# Autodesk Inventor assembly: Assembly
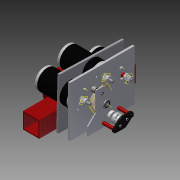
[picture p0: Inventor's stored thumbnail of the model, 180x180]
Saved by Autodesk Inventor 2013 (Build 170138000, 138)
## iProperties
Created: 2013-06-04
Part Number: Assembly
Document SubType Name: Assembly
Designer: mvarma
Author: mvarma
## Documents named in this file (55)
- C:\Users\mvarma\Desktop\GRT 2013-2014 Gearbox\Mark 2\Assembly.iam
- C:\Users\mvarma\Desktop\GRT 2013-2014 Gearbox\Mark 2\Frame Segment.ipt
- C:\Users\mvarma\Desktop\GRT 2013-2014 Gearbox\Mark 2\Plates\Cim Plate.ipt
- C:\Users\mvarma\Desktop\GRT 2013-2014 Gearbox\Mark 2\Wheel Temp.ipt
- C:\Users\mvarma\Desktop\GRT 2013-2014 Gearbox\Mark 2\Motors\Mini CIM Motor.ipt
- C:\Users\mvarma\Desktop\GRT 2013-2014 Gearbox\Mark 2\Motors\CIM Motor.ipt
- C:\Users\mvarma\Desktop\GRT 2013-2014 Gearbox\Mark 2\Pulleys\16T 3mm GT2 - 8mm Key Broach.ipt
- C:\Users\mvarma\Desktop\GRT 2013-2014 Gearbox\Mark 2\Pulleys\48T 3mm GT2 - .375 Hex Broach - Hubless.ipt
- C:\Users\mvarma\Desktop\GRT 2013-2014 Gearbox\Mark 2\Pulleys\56T 3mm GT2 - .375 Hex Broach - Hubless.ipt
- C:\Users\mvarma\Desktop\GRT 2013-2014 Gearbox\Mark 2\Bearings\FR6-2ZZ - Hex.ipt
- C:\Users\mvarma\Desktop\GRT 2013-2014 Gearbox\Mark 2\Spacers\Shim 10 thou .500 Bore.ipt
- C:\Users\mvarma\Desktop\GRT 2013-2014 Gearbox\Mark 2\Shafts\Belt Shaft.ipt
- C:\Users\mvarma\Desktop\GRT 2013-2014 Gearbox\Mark 2\.2500 Spring Clip.ipt
- C:\Users\mvarma\Desktop\GRT 2013-2014 Gearbox\Mark 2\Bearings\R4-2RS.ipt
- C:\Users\mvarma\Desktop\GRT 2013-2014 Gearbox\Mark 2\Spacers\Belt Shaft Spacer 1.ipt
- C:\Users\mvarma\Desktop\GRT 2013-2014 Gearbox\Mark 2\Plates\Pnuematic Plate.ipt
- C:\Users\mvarma\Desktop\GRT 2013-2014 Gearbox\Mark 2\Spacers\Shim 10 thou .375 Bore.ipt
- C:\Users\mvarma\Desktop\GRT 2013-2014 Gearbox\Mark 2\Bearings\FR6-2RS.ipt
- C:\Users\mvarma\Desktop\GRT 2013-2014 Gearbox\Mark 2\Spacers\Belt Shaft Spacer 2.ipt
- C:\Users\mvarma\Desktop\GRT 2013-2014 Gearbox\Mark 2\Shafts\Cluster Shaft.ipt
- C:\Users\mvarma\Desktop\GRT 2013-2014 Gearbox\Mark 2\Gears\15T 20DP - .375 Hex Bore.ipt
- C:\Users\mvarma\Desktop\GRT 2013-2014 Gearbox\Mark 2\Gears\28T 20DP - .375 Hex Bore.ipt
- C:\Users\mvarma\Desktop\GRT 2013-2014 Gearbox\Mark 2\Bearings\FR8-2RS.ipt
- C:\Users\mvarma\Desktop\GRT 2013-2014 Gearbox\Mark 2\Spacers\MiniCim Spacer.ipt
- C:\Users\mvarma\Desktop\GRT 2013-2014 Gearbox\Mark 2\Spacers\Cim Spacer.ipt
- C:\Users\mvarma\Desktop\GRT 2013-2014 Gearbox\Mark 2\Plates\Mounting Plate.ipt
- C:\Users\mvarma\Desktop\GRT 2013-2014 Gearbox\Mark 2\Gears\35T 20DP - .188 Ball Shifting Bore.ipt
- C:\Users\mvarma\Desktop\GRT 2013-2014 Gearbox\Mark 2\Gears\48T 20DP - .188 Ball Shifting Bore.ipt
- C:\Users\mvarma\Desktop\GRT 2013-2014 Gearbox\Mark 2\Bearings\Thrust Bearing Washer - .6250 Bore.ipt
- C:\Users\mvarma\Desktop\GRT 2013-2014 Gearbox\Mark 2\Spacers\Cluster Shaft Spacer.ipt
- C:\Users\mvarma\Desktop\GRT 2013-2014 Gearbox\Mark 2\Bearings\R10-Open.ipt
- C:\Users\mvarma\Desktop\GRT 2013-2014 Gearbox\Mark 2\Bearings\R10-2RS.ipt
- C:\Users\mvarma\Desktop\GRT 2013-2014 Gearbox\Mark 2\Bearing Cover.ipt
- C:\Users\mvarma\Desktop\GRT 2013-2014 Gearbox\Mark 2\Shafts\Output Shaft.ipt
- C:\Users\mvarma\Desktop\GRT 2013-2014 Gearbox\Mark 2\Shafts\Shifting Shaft.ipt
- C:\Users\mvarma\Desktop\GRT 2013-2014 Gearbox\Mark 2\Shafts\Output Shaft Insert.ipt
- C:\Users\mvarma\Desktop\GRT 2013-2014 Gearbox\Mark 2\Ball Bearing 3- 16  in .ipt
- C:\Users\mvarma\Desktop\GRT 2013-2014 Gearbox\Mark 2\Pneumatic\Bore.ipt
- C:\Users\mvarma\Desktop\GRT 2013-2014 Gearbox\Mark 2\Pneumatic\Cylinder.ipt
- C:\Users\mvarma\Desktop\GRT 2013-2014 Gearbox\Mark 2\Pneumatic\Front Mount.ipt
- C:\Users\mvarma\Desktop\GRT 2013-2014 Gearbox\Mark 2\Pneumatic\Rear Mount.ipt
- C:\Users\mvarma\Desktop\GRT 2013-2014 Gearbox\Mark 2\Pneumatic\Shaft.ipt
- C:\Users\mvarma\Desktop\GRT 2013-2014 Gearbox\Mark 2\Pneumatic\Spacer.ipt
- C:\Users\mvarma\Desktop\GRT 2013-2014 Gearbox\Mark 2\Bolts\Socket Head Cap Screw 8-32 Thread .375 Length.ipt
- C:\Users\mvarma\Desktop\GRT 2013-2014 Gearbox\Mark 2\Bolts\Button Head Cap Screw 6-32 Thread .250 Length.ipt
- C:\Users\mvarma\Desktop\GRT 2013-2014 Gearbox\Mark 2\Pneumatic\Pneumatic Connector - Side Side.ipt
- C:\Users\mvarma\Desktop\GRT 2013-2014 Gearbox\Mark 2\Pneumatic\Pneumatic Connector -Actuator Side.ipt
- C:\Users\mvarma\Desktop\GRT 2013-2014 Gearbox\Mark 2\Bolts\Socket Head Cap Screw 8-32 Thread .750 Length.ipt
- C:\Users\mvarma\Desktop\GRT 2013-2014 Gearbox\Mark 2\Bolts\Socket Head Cap Screw 4-40 Thread 1.000 Length.ipt
- C:\Users\mvarma\Desktop\GRT 2013-2014 Gearbox\Mark 2\Spring Pin 1-16 Diameter.ipt
- C:\Users\mvarma\Desktop\GRT 2013-2014 Gearbox\Mark 2\Pneumatic\Mouning Standoff.ipt
- C:\Users\mvarma\Desktop\GRT 2013-2014 Gearbox\Mark 2\Pneumatic\Mounting Insert.ipt
- C:\Users\mvarma\Desktop\GRT 2013-2014 Gearbox\Mark 2\Plates\Pneumatic Mounting Plate.ipt
- C:\Users\mvarma\Desktop\GRT 2013-2014 Gearbox\Mark 2\Pem Nuts\4-40 Clinch Style Pem Nut .091 Minimum Panel Thickness.ipt
- C:\Users\mvarma\Desktop\GRT 2013-2014 Gearbox\Mark 2\Bolts\Socket Head Cap Screw 10-32 Thread 3.000 Length.ipt
## Components (81 placed, 54 different names)
1. Frame Segment:1 — Mate:1, Angle:1, Mate:2, Mate:70, Mate:71
2. Wheel Temp:1 — Mate:2
3. .2500 Spring Clip:1 — Mate:25, Mate:26
4. .2500 Spring Clip:2 — Mate:39, Mate:40
5. Cluster Shaft Spacer:1 — Mate:100, Mate:101
6. R10-2RS:1 — Mate:102, Flush:12
7. Bearing Cover:1 — Mate:106, Mate:107, Mate:108, Mate:160, Mate:161, Mate:162, Mate:163
8. Socket Head Cap Screw 10-32 Thread 3.000 Length:1 — Mate:175, Mate:176
9. Socket Head Cap Screw 10-32 Thread 3.000 Length:2 — Mate:173, Mate:174
10. FR6-2RS:2 — Mate:74, Mate:75, Mate:101
11. FR8-2RS:2 — Mate:72, Mate:73, Mate:99, Flush:13
12. R10-Open:1 — Mate:76, Mate:77, Mate:80, Mate:92, Mate:97, Mate:98
13. R10-Open:2 — Mate:78, Mate:79, Mate:81, Flush:11, Mate:104, Mate:105
14. FR6-2RS:1 — Mate:36, Mate:37, Mate:38, Flush:10
15. FR6-2ZZ - Hex:1 — Mate:19, Mate:20, Angle:3, Mate:22, Mate:44, Mate:96
16. R4-2RS:1 — Mate:27, Mate:28, Mate:29, Flush:9
17. R4-2RS:2 — Mate:27, Mate:28, Mate:42
18. Pneumatic Mounting Plate:1 — Mate:166, Mate:167, Mate:168, Mate:169, Mate:170, Mate:171, Mate:172, Mate:173, Mate:174, Mate:175, Mate:176
19. Mounting Plate:1 — Mate:70, Mate:71, Mate:72, Mate:73, Mate:74, Mate:75
20. Pnuematic Plate:1 — Mate:32, Mate:33, Mate:34, Mate:36, Mate:37, Mate:43
21. Cim Plate:1 — Mate:1, Angle:1, Mate:3, Mate:4, Mate:5, Mate:6, Mate:7, Mate:8, Mate:9, Mate:10, Mate:11, Mate:15, Mate:16, Mate:19, Mate:20, Mate:21, Mate:24, Flush:8, Mate:31, Mate:32, Mate:33, Mate:45, Mate:46, Mate:80, Mate:81, Mate:102, Flush:12, Mate:106, Mate:107, Mate:108, Mate:111
22. 16T 3mm GT2 - 8mm Key Broach:1 — Mate:13, Flush:5, Flush:6
23. 16T 3mm GT2 - 8mm Key Broach:2 — Mate:12, Flush:4, Flush:7
24. 16T 3mm GT2 - 8mm Key Broach:3 — Mate:14, Flush:3, Mate:18
25. 48T 3mm GT2 - .375 Hex Broach - Hubless:1 — Mate:15, Mate:17, Angle:2, Flush:6, Flush:7, Mate:23, Flush:9
26. 56T 3mm GT2 - .375 Hex Broach - Hubless:1 — Mate:16, Mate:17, Angle:2, Mate:18, Angle:3, Mate:35
27. Mini CIM Motor:1 — Mate:3, Mate:4, Mate:5, Mate:14, Flush:3, Mate:51, Mate:52
28. CIM Motor:1 — Mate:9, Mate:10, Mate:11, Mate:12, Flush:4, Mate:53, Mate:54
29. CIM Motor:2 — Mate:6, Mate:7, Mate:8, Mate:13, Flush:5, Mate:55, Mate:56
30. Belt Shaft Spacer 1:1 — Mate:30, Mate:31
31. Belt Shaft Spacer 2:1 — Mate:41, Mate:42
32. MiniCim Spacer:1 — Mate:51, Mate:52
33. Cim Spacer:1 — Mate:53, Mate:54
34. Cim Spacer:2 — Mate:55, Mate:56
35. Shim 10 thou .375 Bore:1 — Mate:34, Mate:35, Mate:38
36. Shim 10 thou .500 Bore:1 — Mate:21, Mate:22, Mate:23
37. Shim 10 thou .500 Bore:2 — Mate:97, Mate:98, Mate:99
38. Thrust Bearing Washer - .6250 Bore:1 — Mate:90, Mate:91, Mate:94
39. Thrust Bearing Washer - .6250 Bore:2 — Mate:90, Mate:91, Mate:92, Mate:93
40. Thrust Bearing Washer - .6250 Bore:3 — Mate:104, Mate:105
41. Belt Shaft:1 — Mate:24, Mate:25, Mate:26, Flush:8, Mate:29, Mate:30, Mate:39, Mate:40, Mate:41
42. Cluster Shaft:1 — Mate:43, Flush:10, Mate:44, Angle:4, Mate:100
43. Output Shaft:1 — Mate:109, Mate:110, Mate:111, Flush:13, Mate:112, Mate:113, Mate:114, Mate:115, Mate:116, Mate:117, Mate:118, Mate:119
44. Shifting Shaft:1 — Mate:109, Mate:110, Transitional:1, Transitional:2, Transitional:3, Transitional:4, Transitional:5, Transitional:6, Mate:135, Flush:16, Mate:158, Flush:17
45. Output Shaft Insert:1 — Mate:112, Mate:113
46. 15T 20DP - .375 Hex Bore:1 — Mate:45, Angle:4, Angle:5, Flush:11, Mate:95, Mate:96
47. 28T 20DP - .375 Hex Bore:1 — Mate:46, Angle:5, Mate:95
48. 35T 20DP - .188 Ball Shifting Bore:1 — Mate:76, Mate:77, Mate:94
49. 48T 20DP - .188 Ball Shifting Bore:1 — Mate:78, Mate:79, Mate:93
50. Ball Bearing 3- 16  in :1 — Mate:116, Transitional:2
51. Ball Bearing 3- 16  in :2 — Mate:114, Transitional:6
52. Ball Bearing 3- 16  in :3 — Mate:115, Transitional:5
53. Ball Bearing 3- 16  in :4 — Mate:117, Transitional:4
54. Ball Bearing 3- 16  in :5 — Mate:119, Transitional:3
55. Ball Bearing 3- 16  in :6 — Mate:118, Transitional:1
56. Bore:1 — Mate:133, Flush:14, Flush:15
57. Cylinder:1 — Mate:130, Mate:131, Mate:132, Flush:15
58. Front Mount:1 — Mate:128, Mate:129, Mate:134, Mate:135, Mate:154, Mate:155, Mate:156, Mate:157
59. Rear Mount:1 — Mate:120, Mate:121, Mate:122, Mate:123, Mate:124, Mate:125, Mate:126, Mate:127, Mate:130, Mate:131, Flush:18, Mate:164, Mate:165, Flush:19, Flush:20, Mate:167
60. Shaft:1 — Mate:132, Mate:133, Flush:14, Mate:138, Mate:139, Mate:140
61. Spacer:1 — Mate:120, Mate:124
62. Spacer:2 — Mate:121, Mate:125, Mate:128
63. Spacer:3 — Mate:122, Mate:126
64. Spacer:4 — Mate:123, Mate:127, Mate:129, Mate:134
65. Socket Head Cap Screw 4-40 Thread 1.000 Length:1 — Mate:155, Mate:157
66. Socket Head Cap Screw 4-40 Thread 1.000 Length:2 — Mate:154, Mate:156
67. Spring Pin 1-16 Diameter:1 — Mate:158, Flush:17
68. Mouning Standoff:1 — Mate:160, Mate:161, Mate:166, Mate:168
69. Mouning Standoff:2 — Mate:162, Mate:163, Flush:18
70. Mounting Insert:1 — Mate:164, Flush:20
71. Mounting Insert:2 — Mate:165, Flush:19
72. 4-40 Clinch Style Pem Nut .091 Minimum Panel Thickness:1 — Mate:169, Mate:170
73. 4-40 Clinch Style Pem Nut .091 Minimum Panel Thickness:2 — Mate:171, Mate:172
74. Socket Head Cap Screw 8-32 Thread .750 Length:2 — Mate:145, Mate:146
75. Socket Head Cap Screw 8-32 Thread .375 Length:1 — Mate:136, Mate:137
76. Button Head Cap Screw 6-32 Thread .250 Length:1 — Mate:152, Mate:153
77. Button Head Cap Screw 6-32 Thread .250 Length:2 — Mate:150, Mate:151
78. Socket Head Cap Screw 8-32 Thread .750 Length:1 — Mate:144, Mate:147
79. R4-2RS:3 — Mate:148, Mate:149, Flush:16
80. Pneumatic Connector - Side Side:1 — Mate:141, Mate:142, Mate:143, Mate:148, Mate:149, Mate:150, Mate:151, Mate:152, Mate:153
81. Pneumatic Connector -Actuator Side:1 — Mate:136, Mate:137, Mate:138, Mate:139, Mate:140, Mate:141, Mate:142, Mate:143, Mate:144, Mate:145, Mate:146, Mate:147
## Relationships (178: Mate 149, Flush 18, Transitional 6, Angle 5)
- Mate:1: Frame Segment:1 ↔ Cim Plate:1
- Angle:1 (0 deg): Frame Segment:1 ↔ Cim Plate:1
- Mate:2: Frame Segment:1 ↔ Wheel Temp:1
- Mate:3: Cim Plate:1 ↔ Mini CIM Motor:1
- Mate:4: Cim Plate:1 ↔ Mini CIM Motor:1
- Mate:5: Cim Plate:1 ↔ Mini CIM Motor:1
- Mate:6: Cim Plate:1 ↔ CIM Motor:2
- Mate:7: Cim Plate:1 ↔ CIM Motor:2
- Mate:8: Cim Plate:1 ↔ CIM Motor:2
- Mate:9: Cim Plate:1 ↔ CIM Motor:1
- Mate:10: Cim Plate:1 ↔ CIM Motor:1
- Mate:11: Cim Plate:1 ↔ CIM Motor:1
- Mate:12: 16T 3mm GT2 - 8mm Key Broach:2 ↔ CIM Motor:1
- Mate:13: 16T 3mm GT2 - 8mm Key Broach:1 ↔ CIM Motor:2
- Mate:14: 16T 3mm GT2 - 8mm Key Broach:3 ↔ Mini CIM Motor:1
- Flush:3: 16T 3mm GT2 - 8mm Key Broach:3 ↔ Mini CIM Motor:1
- Flush:4: 16T 3mm GT2 - 8mm Key Broach:2 ↔ CIM Motor:1
- Flush:5: 16T 3mm GT2 - 8mm Key Broach:1 ↔ CIM Motor:2
- Mate:15: Cim Plate:1 ↔ 48T 3mm GT2 - .375 Hex Broach - Hubless:1
- Mate:16: Cim Plate:1 ↔ 56T 3mm GT2 - .375 Hex Broach - Hubless:1
- Mate:17: 48T 3mm GT2 - .375 Hex Broach - Hubless:1 ↔ 56T 3mm GT2 - .375 Hex Broach - Hubless:1
- Angle:2 (0 deg): 48T 3mm GT2 - .375 Hex Broach - Hubless:1 ↔ 56T 3mm GT2 - .375 Hex Broach - Hubless:1
- Flush:6: 16T 3mm GT2 - 8mm Key Broach:1 ↔ 48T 3mm GT2 - .375 Hex Broach - Hubless:1
- Flush:7: 16T 3mm GT2 - 8mm Key Broach:2 ↔ 48T 3mm GT2 - .375 Hex Broach - Hubless:1
- Mate:18: 16T 3mm GT2 - 8mm Key Broach:3 ↔ 56T 3mm GT2 - .375 Hex Broach - Hubless:1
- Mate:19: FR6-2ZZ - Hex:1 ↔ Cim Plate:1
- Mate:20: FR6-2ZZ - Hex:1 ↔ Cim Plate:1
- Angle:3 (0 deg): FR6-2ZZ - Hex:1 ↔ 56T 3mm GT2 - .375 Hex Broach - Hubless:1
- Mate:21: Cim Plate:1 ↔ Shim 10 thou .500 Bore:1
- Mate:22: FR6-2ZZ - Hex:1 ↔ Shim 10 thou .500 Bore:1
- Mate:23: 48T 3mm GT2 - .375 Hex Broach - Hubless:1 ↔ Shim 10 thou .500 Bore:1
- Mate:24: Cim Plate:1 ↔ Belt Shaft:1
- Mate:25: .2500 Spring Clip:1 ↔ Belt Shaft:1
- Mate:26 (0.0508 mm): .2500 Spring Clip:1 ↔ Belt Shaft:1
- Flush:8: Cim Plate:1 ↔ Belt Shaft:1
- Mate:27: R4-2RS:1 ↔ R4-2RS:2
- Mate:28: R4-2RS:1 ↔ R4-2RS:2
- Mate:29: R4-2RS:1 ↔ Belt Shaft:1
- Flush:9: R4-2RS:1 ↔ 48T 3mm GT2 - .375 Hex Broach - Hubless:1
- Mate:30: Belt Shaft Spacer 1:1 ↔ Belt Shaft:1
- Mate:31: Cim Plate:1 ↔ Belt Shaft Spacer 1:1
- Mate:32: Pnuematic Plate:1 ↔ Cim Plate:1
- Mate:33: Pnuematic Plate:1 ↔ Cim Plate:1
- Mate:34: Pnuematic Plate:1 ↔ Shim 10 thou .375 Bore:1
- Mate:35: 56T 3mm GT2 - .375 Hex Broach - Hubless:1 ↔ Shim 10 thou .375 Bore:1
- Mate:36: FR6-2RS:1 ↔ Pnuematic Plate:1
- Mate:37: FR6-2RS:1 ↔ Pnuematic Plate:1
- Mate:38: FR6-2RS:1 ↔ Shim 10 thou .375 Bore:1
- Mate:39: .2500 Spring Clip:2 ↔ Belt Shaft:1
- Mate:40 (0.0508 mm): .2500 Spring Clip:2 ↔ Belt Shaft:1
- Mate:41: Belt Shaft Spacer 2:1 ↔ Belt Shaft:1
- Mate:42: R4-2RS:2 ↔ Belt Shaft Spacer 2:1
- Mate:43: Pnuematic Plate:1 ↔ Cluster Shaft:1
- Flush:10: FR6-2RS:1 ↔ Cluster Shaft:1
- Mate:44: FR6-2ZZ - Hex:1 ↔ Cluster Shaft:1
- Mate:45: Cim Plate:1 ↔ 15T 20DP - .375 Hex Bore:1
- Mate:46: Cim Plate:1 ↔ 28T 20DP - .375 Hex Bore:1
- Angle:4 (0 deg): Cluster Shaft:1 ↔ 15T 20DP - .375 Hex Bore:1
- Angle:5 (0 deg): 15T 20DP - .375 Hex Bore:1 ↔ 28T 20DP - .375 Hex Bore:1
- Mate:51: Mini CIM Motor:1 ↔ MiniCim Spacer:1
- Mate:52: Mini CIM Motor:1 ↔ MiniCim Spacer:1
- Mate:53: CIM Motor:1 ↔ Cim Spacer:1
- Mate:54: CIM Motor:1 ↔ Cim Spacer:1
- Mate:55: CIM Motor:2 ↔ Cim Spacer:2
- Mate:56: CIM Motor:2 ↔ Cim Spacer:2
- Mate:70: Frame Segment:1 ↔ Mounting Plate:1
- Mate:71: Frame Segment:1 ↔ Mounting Plate:1
- Mate:72: FR8-2RS:2 ↔ Mounting Plate:1
- Mate:73: FR8-2RS:2 ↔ Mounting Plate:1
- Mate:74: FR6-2RS:2 ↔ Mounting Plate:1
- Mate:75: FR6-2RS:2 ↔ Mounting Plate:1
- Mate:76: R10-Open:1 ↔ 35T 20DP - .188 Ball Shifting Bore:1
- Mate:77: R10-Open:1 ↔ 35T 20DP - .188 Ball Shifting Bore:1
- Mate:78: R10-Open:2 ↔ 48T 20DP - .188 Ball Shifting Bore:1
- Mate:79: R10-Open:2 ↔ 48T 20DP - .188 Ball Shifting Bore:1
- Mate:80: R10-Open:1 ↔ Cim Plate:1
- Mate:81: R10-Open:2 ↔ Cim Plate:1
- Mate:90: Thrust Bearing Washer - .6250 Bore:1 ↔ Thrust Bearing Washer - .6250 Bore:2
- Mate:91: Thrust Bearing Washer - .6250 Bore:1 ↔ Thrust Bearing Washer - .6250 Bore:2
- Mate:92: R10-Open:1 ↔ Thrust Bearing Washer - .6250 Bore:2
- Mate:93: Thrust Bearing Washer - .6250 Bore:2 ↔ 48T 20DP - .188 Ball Shifting Bore:1
- Mate:94: Thrust Bearing Washer - .6250 Bore:1 ↔ 35T 20DP - .188 Ball Shifting Bore:1
- Flush:11 (1.5875 mm): R10-Open:2 ↔ 15T 20DP - .375 Hex Bore:1
- Mate:95: 15T 20DP - .375 Hex Bore:1 ↔ 28T 20DP - .375 Hex Bore:1
- Mate:96: FR6-2ZZ - Hex:1 ↔ 15T 20DP - .375 Hex Bore:1
- Mate:97: R10-Open:1 ↔ Shim 10 thou .500 Bore:2
- Mate:98: R10-Open:1 ↔ Shim 10 thou .500 Bore:2
- Mate:99: FR8-2RS:2 ↔ Shim 10 thou .500 Bore:2
- Mate:100: Cluster Shaft Spacer:1 ↔ Cluster Shaft:1
- Mate:101: Cluster Shaft Spacer:1 ↔ FR6-2RS:2
- Mate:102: R10-2RS:1 ↔ Cim Plate:1
- Flush:12: R10-2RS:1 ↔ Cim Plate:1
- Mate:104: R10-Open:2 ↔ Thrust Bearing Washer - .6250 Bore:3
- Mate:105: R10-Open:2 ↔ Thrust Bearing Washer - .6250 Bore:3
- Mate:106: Bearing Cover:1 ↔ Cim Plate:1
- Mate:107: Bearing Cover:1 ↔ Cim Plate:1
- Mate:108: Bearing Cover:1 ↔ Cim Plate:1
- Mate:109: Output Shaft:1 ↔ Shifting Shaft:1
- Mate:110 (3.175 mm): Output Shaft:1 ↔ Shifting Shaft:1
- Mate:111: Cim Plate:1 ↔ Output Shaft:1
- Flush:13: FR8-2RS:2 ↔ Output Shaft:1
- Mate:112: Output Shaft:1 ↔ Output Shaft Insert:1
- Mate:113: Output Shaft:1 ↔ Output Shaft Insert:1
- Mate:114: Output Shaft:1 ↔ Ball Bearing 3- 16  in :2
- Mate:115: Output Shaft:1 ↔ Ball Bearing 3- 16  in :3
- Mate:116: Output Shaft:1 ↔ Ball Bearing 3- 16  in :1
- Mate:117: Output Shaft:1 ↔ Ball Bearing 3- 16  in :4
- Mate:118: Output Shaft:1 ↔ Ball Bearing 3- 16  in :6
- Mate:119: Output Shaft:1 ↔ Ball Bearing 3- 16  in :5
- Transitional:1: Shifting Shaft:1 ↔ Ball Bearing 3- 16  in :6
- Transitional:2: Shifting Shaft:1 ↔ Ball Bearing 3- 16  in :1
- Transitional:3: Shifting Shaft:1 ↔ Ball Bearing 3- 16  in :5
- Transitional:4: Shifting Shaft:1 ↔ Ball Bearing 3- 16  in :4
- Transitional:5: Shifting Shaft:1 ↔ Ball Bearing 3- 16  in :3
- Transitional:6: Shifting Shaft:1 ↔ Ball Bearing 3- 16  in :2
- Mate:120: Rear Mount:1 ↔ Spacer:1
- Mate:121: Rear Mount:1 ↔ Spacer:2
- Mate:122: Rear Mount:1 ↔ Spacer:3
- Mate:123: Rear Mount:1 ↔ Spacer:4
- Mate:124: Rear Mount:1 ↔ Spacer:1
- Mate:125: Rear Mount:1 ↔ Spacer:2
- Mate:126: Rear Mount:1 ↔ Spacer:3
- Mate:127: Rear Mount:1 ↔ Spacer:4
- Mate:128: Front Mount:1 ↔ Spacer:2
- Mate:129: Front Mount:1 ↔ Spacer:4
- Mate:130: Cylinder:1 ↔ Rear Mount:1
- Mate:131: Cylinder:1 ↔ Rear Mount:1
- Mate:132: Cylinder:1 ↔ Shaft:1
- Mate:133: Bore:1 ↔ Shaft:1
- Flush:14: Bore:1 ↔ Shaft:1
- Flush:15: Bore:1 ↔ Cylinder:1
- Mate:134: Front Mount:1 ↔ Spacer:4
- Mate:135: Shifting Shaft:1 ↔ Front Mount:1
- Mate:136: Socket Head Cap Screw 8-32 Thread .375 Length:1 ↔ Pneumatic Connector -Actuator Side:1
- Mate:137: Socket Head Cap Screw 8-32 Thread .375 Length:1 ↔ Pneumatic Connector -Actuator Side:1
- Mate:138: Shaft:1 ↔ Pneumatic Connector -Actuator Side:1
- Mate:139: Shaft:1 ↔ Pneumatic Connector -Actuator Side:1
- Mate:140: Shaft:1 ↔ Pneumatic Connector -Actuator Side:1
- Mate:141: Pneumatic Connector - Side Side:1 ↔ Pneumatic Connector -Actuator Side:1
- Mate:142: Pneumatic Connector - Side Side:1 ↔ Pneumatic Connector -Actuator Side:1
- Mate:143: Pneumatic Connector - Side Side:1 ↔ Pneumatic Connector -Actuator Side:1
- Mate:144: Socket Head Cap Screw 8-32 Thread .750 Length:1 ↔ Pneumatic Connector -Actuator Side:1
- Mate:145: Socket Head Cap Screw 8-32 Thread .750 Length:2 ↔ Pneumatic Connector -Actuator Side:1
- Mate:146: Socket Head Cap Screw 8-32 Thread .750 Length:2 ↔ Pneumatic Connector -Actuator Side:1
- Mate:147: Socket Head Cap Screw 8-32 Thread .750 Length:1 ↔ Pneumatic Connector -Actuator Side:1
- Mate:148: R4-2RS:3 ↔ Pneumatic Connector - Side Side:1
- Mate:149: R4-2RS:3 ↔ Pneumatic Connector - Side Side:1
- Mate:150: Button Head Cap Screw 6-32 Thread .250 Length:2 ↔ Pneumatic Connector - Side Side:1
- Mate:151: Button Head Cap Screw 6-32 Thread .250 Length:2 ↔ Pneumatic Connector - Side Side:1
- Mate:152: Button Head Cap Screw 6-32 Thread .250 Length:1 ↔ Pneumatic Connector - Side Side:1
- Mate:153: Button Head Cap Screw 6-32 Thread .250 Length:1 ↔ Pneumatic Connector - Side Side:1
- Mate:154: Front Mount:1 ↔ Socket Head Cap Screw 4-40 Thread 1.000 Length:2
- Mate:155: Front Mount:1 ↔ Socket Head Cap Screw 4-40 Thread 1.000 Length:1
- Mate:156: Front Mount:1 ↔ Socket Head Cap Screw 4-40 Thread 1.000 Length:2
- Mate:157: Front Mount:1 ↔ Socket Head Cap Screw 4-40 Thread 1.000 Length:1
- Flush:16 (-2.54 mm): Shifting Shaft:1 ↔ R4-2RS:3
- Mate:158: Shifting Shaft:1 ↔ Spring Pin 1-16 Diameter:1
- Flush:17: Shifting Shaft:1 ↔ Spring Pin 1-16 Diameter:1
- Mate:160: Bearing Cover:1 ↔ Mouning Standoff:1
- Mate:161: Bearing Cover:1 ↔ Mouning Standoff:1
- Mate:162: Bearing Cover:1 ↔ Mouning Standoff:2
- Mate:163: Bearing Cover:1 ↔ Mouning Standoff:2
- Flush:18: Rear Mount:1 ↔ Mouning Standoff:2
- Mate:164: Rear Mount:1 ↔ Mounting Insert:1
- Mate:165: Rear Mount:1 ↔ Mounting Insert:2
- Flush:19: Rear Mount:1 ↔ Mounting Insert:2
- Flush:20: Rear Mount:1 ↔ Mounting Insert:1
- Mate:166: Pneumatic Mounting Plate:1 ↔ Mouning Standoff:1
- Mate:167: Pneumatic Mounting Plate:1 ↔ Rear Mount:1
- Mate:168: Pneumatic Mounting Plate:1 ↔ Mouning Standoff:1
- Mate:169: Pneumatic Mounting Plate:1 ↔ 4-40 Clinch Style Pem Nut .091 Minimum Panel Thickness:1
- Mate:170: Pneumatic Mounting Plate:1 ↔ 4-40 Clinch Style Pem Nut .091 Minimum Panel Thickness:1
- Mate:171: Pneumatic Mounting Plate:1 ↔ 4-40 Clinch Style Pem Nut .091 Minimum Panel Thickness:2
- Mate:172: Pneumatic Mounting Plate:1 ↔ 4-40 Clinch Style Pem Nut .091 Minimum Panel Thickness:2
- Mate:173: Socket Head Cap Screw 10-32 Thread 3.000 Length:2 ↔ Pneumatic Mounting Plate:1
- Mate:174: Socket Head Cap Screw 10-32 Thread 3.000 Length:2 ↔ Pneumatic Mounting Plate:1
- Mate:175: Socket Head Cap Screw 10-32 Thread 3.000 Length:1 ↔ Pneumatic Mounting Plate:1
- Mate:176: Socket Head Cap Screw 10-32 Thread 3.000 Length:1 ↔ Pneumatic Mounting Plate:1
